# Autodesk Inventor assembly: ASSEMBLY_pring
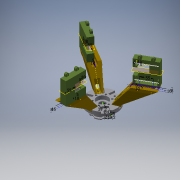
[picture p0: Inventor's stored thumbnail of the model, 180x180]
Saved by Autodesk Inventor 2018 (Build 220112000, 112)
## iProperties
Created: 2026-06-13
Part Number: ASSEMBLY_pring
Document SubType Name: Assembly
Designer: neo
Author: neo
## Documents named in this file (6)
- C:\Users\neo\Documents\neoatlantis-shared\projects\kreion\design2\ASSEMBLY_pring.iam
- C:\Users\neo\Documents\neoatlantis-shared\projects\kreion\design2\PRING_terminal-cap.ipt
- C:\Users\neo\Documents\neoatlantis-shared\projects\kreion\design2\ASSEMBLY_pring_vbar_holder.iam
- C:\Users\neo\Documents\neoatlantis-shared\projects\kreion\design2\HELP_6204BEARING_CASE_A.ipt
- C:\Users\neo\Documents\neoatlantis-shared\projects\kreion\design2\HELP_6204BEARING_CASE_B.ipt
- C:\Users\neo\Documents\neoatlantis-shared\projects\kreion\design2\PRING_piston.ipt
## Components (7 placed, 5 different names)
1. PRING_terminal-cap:1 — Mate:1, Tangent:1, Mate:2, Insert:1, Tangent:2
2. HELP_6204BEARING_CASE_A:1 — Mate:2, Insert:1, Tangent:2, Insert:2, Tangent:3
3. HELP_6204BEARING_CASE_B:1 — Insert:2, Tangent:3
4. PRING_piston:1 — Tangent:4, Tangent:5, Tangent:6
5. ASSEMBLY_pring_vbar_holder:1 [sub-assembly] — Mate:1, Tangent:1, Tangent:4, Tangent:5, Tangent:6
6. ASSEMBLY_pring_vbar_holder:2 [sub-assembly]
7. ASSEMBLY_pring_vbar_holder:3 [sub-assembly]
## Component patterns: (3 elements, first: ASSEMBLY_pring_vbar_holder:1)
## Relationships (10: Tangent 6, Mate 2, Insert 2)
- Mate:1: PRING_terminal-cap:1 ↔ ASSEMBLY_pring_vbar_holder:1
- Tangent:1: PRING_terminal-cap:1 ↔ ASSEMBLY_pring_vbar_holder:1
- Mate:2: PRING_terminal-cap:1 ↔ HELP_6204BEARING_CASE_A:1
- Insert:1: PRING_terminal-cap:1 ↔ HELP_6204BEARING_CASE_A:1
- Tangent:2: PRING_terminal-cap:1 ↔ HELP_6204BEARING_CASE_A:1
- Insert:2: HELP_6204BEARING_CASE_A:1 ↔ HELP_6204BEARING_CASE_B:1
- Tangent:3: HELP_6204BEARING_CASE_A:1 ↔ HELP_6204BEARING_CASE_B:1
- Tangent:4: PRING_piston:1 ↔ ASSEMBLY_pring_vbar_holder:1
- Tangent:5: PRING_piston:1 ↔ ASSEMBLY_pring_vbar_holder:1
- Tangent:6: PRING_piston:1 ↔ ASSEMBLY_pring_vbar_holder:1
